# Autodesk Inventor assembly: photodetector_assembly
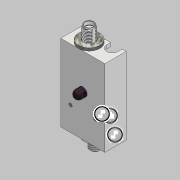
[picture p0: Inventor's stored thumbnail of the model, 180x180]
Saved by Autodesk Inventor 2021.4 (Build 254397000, 397)
## iProperties
Created: 2022-11-02
Part Number: photodetector_assembly
Document SubType Name: Assembly
Designer: Tilman Preuschoff
Author: Tilman Preuschoff
## Documents named in this file (7)
- C:\Users\Tilman Preuschoff\Documents\GitHub\SFH203_photodetector\case\assembly\photodetector_assembly.iam
- C:\Users\Tilman Preuschoff\Documents\GitHub\SFH203_photodetector\case\case.ipt
- C:\Users\Tilman Preuschoff\Documents\GitHub\SFH203_photodetector\case\assembly\SFH203_photodetector.iam
- C:\Users\Tilman Preuschoff\Documents\Inventor\Content Center Files\R2021\de-DE\DIN 84\DIN 84 - M2,5 x 5.ipt
- C:\Users\Tilman Preuschoff\Documents\Inventor\Content Center Files\R2021\de-DE\DIN 125-1  A\DIN 125 - A 6,4.ipt
- C:\Users\Tilman Preuschoff\Documents\Inventor\Content Center Files\R2021\de-DE\DIN 914\DIN 914 - M6 x 16.ipt
- C:\Users\Tilman Preuschoff\Documents\GitHub\SFH203_photodetector\case\cover.ipt
## Components (9 placed, 6 different names)
1. case:1 — Passend:1, Passend:3, Winkel:1, Drehbar:5, Starr:1, Passend:5, Passend:7, Winkel:3, Passend:8, Passend:9, Winkel:4, Passend:10, Passend:11
2. DIN 84 - ersetzt durch DIN EN ISO 1207 M2,5 x 5:3
3. DIN 84 - ersetzt durch DIN EN ISO 1207 M2,5 x 5:4
4. DIN 125-1 A A 6,4:1 — Starr:1
5. DIN 914 M6 x 16:1 — Drehbar:5
6. DIN 125-1 A A 6,4:2 — Passend:5
7. cover:1 — Passend:7, Winkel:3, Passend:8
8. SFH203_photodetector:1 [sub-assembly] — Passend:9, Winkel:4, Passend:10
9. DIN 125-1 A A 6,4:3 — Passend:11
## Relationships (13: Mate 8, Angle 3, RevoluteJoint 1, WeldJoint 1)
- Passend:1 [Mate]: case:1
- Passend:3 [Mate]: case:1
- Winkel:1 [Angle] (0 deg): case:1
- Drehbar:5 [RevoluteJoint] (6 mm): case:1 ↔ DIN 914 M6 x 16:1
- Starr:1 [WeldJoint]: case:1 ↔ DIN 125-1 A A 6,4:1
- Passend:5 [Mate]: case:1 ↔ DIN 125-1 A A 6,4:2
- Passend:7 [Mate]: case:1 ↔ cover:1
- Winkel:3 [Angle] (180 deg): case:1 ↔ cover:1
- Passend:8 [Mate]: case:1 ↔ cover:1
- Passend:9 [Mate]: case:1 ↔ SFH203_photodetector:1
- Winkel:4 [Angle] (180 deg): case:1 ↔ SFH203_photodetector:1
- Passend:10 [Mate]: case:1 ↔ SFH203_photodetector:1
- Passend:11 [Mate]: case:1 ↔ DIN 125-1 A A 6,4:3
